# Autodesk Inventor assembly: flute
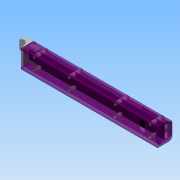
[picture p0: Inventor's stored thumbnail of the model, 180x180]
Saved by Autodesk Inventor 2015 (Build 190159000, 159)
## iProperties
Created: 2016-04-17
Part Number: flute
Document SubType Name: Assembly
Designer: Gregwar
Author: Gregwar
## Documents named in this file (10)
- C:\Users\Gregwar\Desktop\eFlute\3d\v1.2\flute.iam
- C:\Users\Gregwar\Desktop\eFlute\3d\v1.2\electronics.ipt
- C:\Users\Gregwar\Desktop\eFlute\3d\v1.2\top.ipt
- C:\Users\Gregwar\Desktop\eFlute\3d\v1.2\entretoise_6.ipt
- C:\Users\Gregwar\Desktop\eFlute\3d\v1.2\entretoise_8.ipt
- C:\Users\Gregwar\Desktop\eFlute\3d\v1.2\bottom.ipt
- C:\Users\Gregwar\Desktop\eFlute\3d\v1.2\connectors.ipt
- C:\Users\Gregwar\Desktop\eFlute\3d\v1.2\mouthpiece.ipt
- C:\Users\Gregwar\Desktop\eFlute\3d\v1.2\fraisee.ipt
- C:\Users\Gregwar\Desktop\eFlute\3d\v1.2\fraisee_MIR.ipt
## Components (37 placed, 9 different names)
1. electronics:1 — Placage:1, Placage:2, Placage:3, Placage:4, Placage:5, Placage:7, Placage:8, Placage:9, Placage:10, Placage:11, Placage:12, Placage:13, Placage:14, Placage:15, Placage:16, Placage:17, Placage:18, Placage:19, Placage:20, Placage:21, Placage:22, Placage:23, Placage:24, Placage:25, Placage:26, Placage:27, Placage:28, Placage:29, Placage:30, Placage:31, Placage:32, Placage:40
2. top:1 — Placage:33, Placage:34, Placage:35, Affleurement:1, Placage:41, Placage:42, Placage:43, Placage:44, Affleurement:2, Placage:45, Affleurement:3, Placage:46, Affleurement:4, Placage:47, Affleurement:5, Placage:48, Affleurement:6, Placage:49, Affleurement:7, Placage:50, Affleurement:8, Placage:51, Affleurement:9, Placage:52, Symétrie:1
3. entretoise_6:1 — Placage:1, Placage:2, Placage:6, Placage:34
4. entretoise_6:2 — Placage:3, Placage:4, Placage:35
5. entretoise_6:3 — Placage:5, Placage:6, Placage:38
6. entretoise_6:4 — Placage:7, Placage:8, Placage:37
7. entretoise_8:1 — Placage:9, Placage:10
8. entretoise_8:2 — Placage:11, Placage:12
9. entretoise_8:3 — Placage:13, Placage:14
10. entretoise_8:4 — Placage:15, Placage:16, Placage:39
11. entretoise_8:5 — Placage:17, Placage:18
12. entretoise_8:6 — Placage:19, Placage:20
13. entretoise_8:7 — Placage:21, Placage:22
14. entretoise_8:8 — Placage:23, Placage:24
15. entretoise_8:9 — Placage:25, Placage:26
16. entretoise_8:10 — Placage:27, Placage:28
17. entretoise_8:11 — Placage:29, Placage:30, Placage:33
18. entretoise_8:12 — Placage:31, Placage:32
19. bottom:1 — Placage:37, Placage:38, Placage:39, Symétrie:1
20. connectors:1 — Placage:40, Affleurement:1, Placage:41
21. mouthpiece:1 — Placage:42, Placage:43, Placage:44
22. fraisee:1 — Affleurement:2, Placage:45
23. fraisee:2 — Affleurement:3, Placage:46
24. fraisee:3 — Affleurement:4, Placage:47
25. fraisee:4 — Affleurement:5, Placage:48
26. fraisee:5 — Affleurement:6, Placage:49
27. fraisee:6 — Affleurement:7, Placage:50
28. fraisee:7 — Affleurement:8, Placage:51
29. fraisee:8 — Affleurement:9, Placage:52
30. fraisee_MIR:1
31. fraisee_MIR:2
32. fraisee_MIR:3
33. fraisee_MIR:4
34. fraisee_MIR:5
35. fraisee_MIR:6
36. fraisee_MIR:7
37. fraisee_MIR:8
## Relationships (61: Mate 51, Flush 9, Symmetry 1)
- Placage:1 [Mate]: electronics:1 ↔ entretoise_6:1
- Placage:2 [Mate]: electronics:1 ↔ entretoise_6:1
- Placage:3 [Mate]: electronics:1 ↔ entretoise_6:2
- Placage:4 [Mate]: electronics:1 ↔ entretoise_6:2
- Placage:5 [Mate]: electronics:1 ↔ entretoise_6:3
- Placage:6 [Mate]: entretoise_6:1 ↔ entretoise_6:3
- Placage:7 [Mate]: electronics:1 ↔ entretoise_6:4
- Placage:8 [Mate]: electronics:1 ↔ entretoise_6:4
- Placage:9 [Mate]: electronics:1 ↔ entretoise_8:1
- Placage:10 [Mate]: electronics:1 ↔ entretoise_8:1
- Placage:11 [Mate]: electronics:1 ↔ entretoise_8:2
- Placage:12 [Mate]: electronics:1 ↔ entretoise_8:2
- Placage:13 [Mate]: electronics:1 ↔ entretoise_8:3
- Placage:14 [Mate]: electronics:1 ↔ entretoise_8:3
- Placage:15 [Mate]: electronics:1 ↔ entretoise_8:4
- Placage:16 [Mate]: electronics:1 ↔ entretoise_8:4
- Placage:17 [Mate]: electronics:1 ↔ entretoise_8:5
- Placage:18 [Mate]: electronics:1 ↔ entretoise_8:5
- Placage:19 [Mate]: electronics:1 ↔ entretoise_8:6
- Placage:20 [Mate]: electronics:1 ↔ entretoise_8:6
- Placage:21 [Mate]: electronics:1 ↔ entretoise_8:7
- Placage:22 [Mate]: electronics:1 ↔ entretoise_8:7
- Placage:23 [Mate]: electronics:1 ↔ entretoise_8:8
- Placage:24 [Mate]: electronics:1 ↔ entretoise_8:8
- Placage:25 [Mate]: electronics:1 ↔ entretoise_8:9
- Placage:26 [Mate]: electronics:1 ↔ entretoise_8:9
- Placage:27 [Mate]: electronics:1 ↔ entretoise_8:10
- Placage:28 [Mate]: electronics:1 ↔ entretoise_8:10
- Placage:29 [Mate]: electronics:1 ↔ entretoise_8:11
- Placage:30 [Mate]: electronics:1 ↔ entretoise_8:11
- Placage:31 [Mate]: electronics:1 ↔ entretoise_8:12
- Placage:32 [Mate]: electronics:1 ↔ entretoise_8:12
- Placage:33 [Mate]: top:1 ↔ entretoise_8:11
- Placage:34 [Mate]: top:1 ↔ entretoise_6:1
- Placage:35 [Mate]: top:1 ↔ entretoise_6:2
- Placage:37 [Mate]: entretoise_6:4 ↔ bottom:1
- Placage:38 [Mate]: entretoise_6:3 ↔ bottom:1
- Placage:39 [Mate]: entretoise_8:4 ↔ bottom:1
- Placage:40 [Mate]: electronics:1 ↔ connectors:1
- Affleurement:1 [Flush]: top:1 ↔ connectors:1
- Placage:41 [Mate]: top:1 ↔ connectors:1
- Placage:42 [Mate]: top:1 ↔ mouthpiece:1
- Placage:43 [Mate]: top:1 ↔ mouthpiece:1
- Placage:44 [Mate]: top:1 ↔ mouthpiece:1
- Affleurement:2 [Flush]: top:1 ↔ fraisee:1
- Placage:45 [Mate]: top:1 ↔ fraisee:1
- Affleurement:3 [Flush]: top:1 ↔ fraisee:2
- Placage:46 [Mate]: top:1 ↔ fraisee:2
- Affleurement:4 [Flush]: top:1 ↔ fraisee:3
- Placage:47 [Mate]: top:1 ↔ fraisee:3
- Affleurement:5 [Flush]: top:1 ↔ fraisee:4
- Placage:48 [Mate]: top:1 ↔ fraisee:4
- Affleurement:6 [Flush]: top:1 ↔ fraisee:5
- Placage:49 [Mate]: top:1 ↔ fraisee:5
- Affleurement:7 [Flush]: top:1 ↔ fraisee:6
- Placage:50 [Mate]: top:1 ↔ fraisee:6
- Affleurement:8 [Flush]: top:1 ↔ fraisee:7
- Placage:51 [Mate]: top:1 ↔ fraisee:7
- Affleurement:9 [Flush]: top:1 ↔ fraisee:8
- Placage:52 [Mate]: top:1 ↔ fraisee:8
- Symétrie:1 [Symmetry]: top:1 ↔ bottom:1
